# Autodesk Inventor assembly: 539636 HGP-16-A-B-SSK---(asm_0_-ZH)
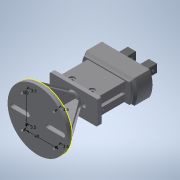
[picture p0: Inventor's stored thumbnail of the model, 180x180]
Saved by Autodesk Inventor 2021 (Build 250183000, 183)
## iProperties
Category: PARTsolutions
Company: FESTO
Created: 2023-03-06
Part Number: 539636 HGP-16-A-B-SSK---(asm_0_-ZH)
Catalog Web Link: www.cadenas.de
Description: HGP-parallel gripper
Vendor: FESTO
Document SubType Name: Assembly
Designer: psAdmin
Manufacturer: FESTO
Mass: 197 g
Surface Area: 188.34 cm^2
Volume: 85.0261 cm^3
Density: 2.31694 g/cm^3
PSOL_IDENT_0: {$CADENAS_DATA/23d-libs/festo/parts/h/hgp/hgp_asm_tab.prj},226 {VTYP=3D},{STYP=ASSTAB},{NB=539636 HG
PSOL_IDENT_1: P-16-A-B-SSK---(asm_0_-ZH)},{LINA=539636 HGP-16-A-B-SSK},{NN=HGP},{DATE=10.09.2021 08:18:21},{GEOMDA
PSOL_IDENT_2: TE=23.06.2021 10:05:29},{VERSION=},{LINEID=210},{WBVAR=HUBST,ZBH},{WBNUMERIC=HUBST,ZBH}  {NB=539636
PSOL_IDENT_3: HGP-16-A-B-SSK---(asm_0_-ZH)},{LINA=539636 HGP-16-A-B-SSK},{KT=3},{TNR=539636},{TYP=HGP-16-A-B-SSK},
PSOL_IDENT_4: {INFO=},{EOLDATE=},{KDM=16},{HUBST=0},{ZBH=1},{B1=47.000},{B2=25.000},{B3=16.400},{B4=26.400},{B5=46
PSOL_IDENT_5: .400},{B6=10.000},{D2=M 4},{D3=7.000},{D4=M 4},{D5=3.300},{D6=3.000},{EE=M 3},{H1=83.000},{H2=20.500
PSOL_IDENT_6: },{H3=21.900},{H4=7.500},{H5=7.000},{H6=4.000},{H7=11.000},{H8=5.500},{H9=10.000},{L1=22.000},{L2=5.
PSOL_IDENT_7: 700},{L3=10.000},{L6=0.000},{T1=1.600},{T2=7.000},{T3=8.000},{T4=3.500},{T5=1.400},{EEP=3.000},{KDRE
PSOL_IDENT_8: E=2.459},{D2P=4.000},{KDR2=3.242},{D4P=4.000},{KDR5=3.242},{LHUB=5.000},{VERS=3.000},{ZT=-ZH},{PPATH=
PSOL_IDENT_9: assemblies/hgp_sbl.prj},{VIS=1},{CNSMASSEXACT=0.197}
NB: 539636 HGP-16-A-B-SSK---(asm_0_-ZH)
NN: HGP
NT: parallel gripper
NBSYN: $TNR. $TYP.---(asm_$HUBST._$ZT.)
LINA: 539636 HGP-16-A-B-SSK
CATALOG: Festo
TNR: 539636
TYP: HGP-16-A-B-SSK
HUBST: 0
ZBH: With centring sleeves (2xZBH)
B1: 47
B2: 25
B3: 16.4
B4: 26.4
B5: 46.4
B6: 10
D2: M 4
D3: 7
D4: M 4
D5: 3.3
D6: 3
EE: M 3
H1: 83
H2: 20.5
H3: 21.9
H4: 7.5
H5: 7
H6: 4
H7: 11
H8: 5.5
H9: 10
L1: 22
L2: 5.7
L3: 10
L6: 0
T1: 1.6
T2: 7
T3: 8
T4: 3.5
T5: 1.4
D4P: 4
CNSMASSEXACT: 0.197
SUPPLIER: FESTO
ARTICLENO: 539636 HGP-16-A-B-SSK---(asm_0_-ZH)
BOMINFO: 539636 HGP-16-A-B-SSK
CREATOR: CADENAS GmbH
Title: 539636 HGP-16-A-B-SSK
Author: Cadenas PARTsolutions
Comments: parallel gripper
## Documents named in this file (4)
- D:\AsU\semesters\senior 2\new_gripper\3dfindit-Festo-539636_HGP-16-A-B-SSK---_asm_0_-ZH_-0202303061711339323165410e898ce\AIS2021\539636 HGP-16-A-B-SSK---(asm_0_-ZH).iam
- D:\AsU\semesters\senior 2\new_gripper\3dfindit-Festo-539636_HGP-16-A-B-SSK---_asm_0_-ZH_-0202303061711339323165410e898ce\AIS2021\539636 HGP-16-A-B-SSK---(0_1_ZYL).ipt
- D:\AsU\semesters\senior 2\new_gripper\3dfindit-Festo-539636_HGP-16-A-B-SSK---_asm_0_-ZH_-0202303061711339323165410e898ce\AIS2021\HGP-16---(116_JAW).ipt
- D:\AsU\semesters\senior 2\new_gripper\gripper extension.ipt
## Components (4 placed, 3 different names)
1. 539636 HGP-16-A-B-SSK---(0_1_ZYL):1 — JAW_1_XY@1 <-> ANBAU_XY@4, JAW_1_Z@1 <-> ANBAU_Z@4, JAW_1_YZ@1 <-> ANBAU_YZ@4, JAW_2_XY@1 <-> ANBAU_XY@5, JAW_2_Z@1 <-> ANBAU_Z@5, JAW_2_YZ@1 <-> ANBAU_YZ@5, Mate:9
2. HGP-16---(116_JAW):1 — JAW_1_XY@1 <-> ANBAU_XY@4, JAW_1_Z@1 <-> ANBAU_Z@4, JAW_1_YZ@1 <-> ANBAU_YZ@4
3. HGP-16---(116_JAW):2 — JAW_2_XY@1 <-> ANBAU_XY@5, JAW_2_Z@1 <-> ANBAU_Z@5, JAW_2_YZ@1 <-> ANBAU_YZ@5
4. gripper extension:1 — Mate:9
## Relationships (7: Mate 5, Angle 2)
- JAW_1_XY@1 <-> ANBAU_XY@4 [Mate]: 539636 HGP-16-A-B-SSK---(0_1_ZYL):1 ↔ HGP-16---(116_JAW):1
- JAW_1_Z@1 <-> ANBAU_Z@4 [Mate]: 539636 HGP-16-A-B-SSK---(0_1_ZYL):1 ↔ HGP-16---(116_JAW):1
- JAW_1_YZ@1 <-> ANBAU_YZ@4 [Angle] (0 deg): 539636 HGP-16-A-B-SSK---(0_1_ZYL):1 ↔ HGP-16---(116_JAW):1
- JAW_2_XY@1 <-> ANBAU_XY@5 [Mate]: 539636 HGP-16-A-B-SSK---(0_1_ZYL):1 ↔ HGP-16---(116_JAW):2
- JAW_2_Z@1 <-> ANBAU_Z@5 [Mate]: 539636 HGP-16-A-B-SSK---(0_1_ZYL):1 ↔ HGP-16---(116_JAW):2
- JAW_2_YZ@1 <-> ANBAU_YZ@5 [Angle] (0 deg): 539636 HGP-16-A-B-SSK---(0_1_ZYL):1 ↔ HGP-16---(116_JAW):2
- Mate:9: 539636 HGP-16-A-B-SSK---(0_1_ZYL):1 ↔ gripper extension:1
